# Autodesk Inventor assembly: Apparaten
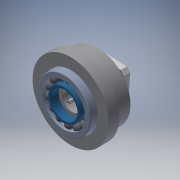
[picture p0: Inventor's stored thumbnail of the model, 180x180]
Saved by Autodesk Inventor 2016 (Build 200138000, 138)
## iProperties
Created: 2018-01-17
Part Number: Apparaten
Document SubType Name: Assembly
Designer: John
Author: John
## Documents named in this file (4)
- C:\Users\John\Killemall\Apparaten.iam
- C:\Users\John\Killemall\FAG\inafag_7208-b-xl-tvp_4yn0b4tr5qy7sto7dos6bxdjs.iam
- C:\Users\John\Killemall\Motor\M1173041- NEMA 17.ipt
- C:\Users\John\Documents\Part1.ipt
## Components (3 placed, 3 different names)
1. inafag_7208-b-xl-tvp_4yn0b4tr5qy7sto7dos6bxdjs:1 [sub-assembly] — Mate:4, Mate:6, Mate:7
2. Part1:1 — Mate:5, Mate:6, Mate:7
3. M1173041- NEMA 17:1 — Mate:4, Mate:5
## Relationships (4: Mate 4)
- Mate:4: inafag_7208-b-xl-tvp_4yn0b4tr5qy7sto7dos6bxdjs:1 ↔ M1173041- NEMA 17:1
- Mate:5: Part1:1 ↔ M1173041- NEMA 17:1
- Mate:6: inafag_7208-b-xl-tvp_4yn0b4tr5qy7sto7dos6bxdjs:1 ↔ Part1:1
- Mate:7: inafag_7208-b-xl-tvp_4yn0b4tr5qy7sto7dos6bxdjs:1 ↔ Part1:1
